# Autodesk Inventor assembly: Second Case
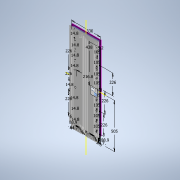
[picture p0: Inventor's stored thumbnail of the model, 180x180]
Saved by Autodesk Inventor 2021 (Build 250183000, 183)
## iProperties
Created: 2022-02-06
Part Number: Second Case
Document SubType Name: Assembly
Designer: tlar613
Author: tlar613
## Documents named in this file (6)
- \\unifiles.uoa.auckland.ac.nz\myhome\Documents\GitHub\2021_SRW_RC_CAR\Magnetics\Final Coil Design\CadModels\SecondCasing\Second Case.iam
- \\unifiles.uoa.auckland.ac.nz\myhome\Documents\GitHub\2021_SRW_RC_CAR\Magnetics\Final Coil Design\CadModels\SecondCasing\Base.ipt
- \\unifiles.uoa.auckland.ac.nz\myhome\Documents\GitHub\2021_SRW_RC_CAR\Magnetics\Final Coil Design\CadModels\SecondCasing\AluminumCasing.ipt
- \\unifiles.uoa.auckland.ac.nz\myhome\Documents\GitHub\2021_SRW_RC_CAR\Magnetics\Final Coil Design\CadModels\SecondCasing\AluminumSheet.ipt
- \\unifiles.uoa.auckland.ac.nz\myhome\Documents\GitHub\2021_SRW_RC_CAR\Magnetics\Final Coil Design\CadModels\SecondCasing\FerriteLayer.ipt
- \\unifiles.uoa.auckland.ac.nz\myhome\Documents\GitHub\2021_SRW_RC_CAR\Magnetics\Final Coil Design\CadModels\SecondCasing\CoilCasing.ipt
## Components (5 placed, 5 different names)
1. Base:1 — Mate:1, Mate:2, Flush:13, Flush:14
2. AluminumCasing:1 — Mate:1, Mate:4, Mate:5, Mate:7, Flush:12, Flush:13, Flush:14
3. AluminumSheet:1 — Mate:2, Mate:4, Mate:7
4. FerriteLayer:1 — Mate:5
5. CoilCasing:1 — Flush:12
## Relationships (8: Mate 5, Flush 3)
- Mate:1: Base:1 ↔ AluminumCasing:1
- Mate:2: Base:1 ↔ AluminumSheet:1
- Mate:4: AluminumCasing:1 ↔ AluminumSheet:1
- Mate:5: AluminumCasing:1 ↔ FerriteLayer:1
- Mate:7: AluminumCasing:1 ↔ AluminumSheet:1
- Flush:12: AluminumCasing:1 ↔ CoilCasing:1
- Flush:13: Base:1 ↔ AluminumCasing:1
- Flush:14: Base:1 ↔ AluminumCasing:1
